# Autodesk Inventor assembly: Assembly7
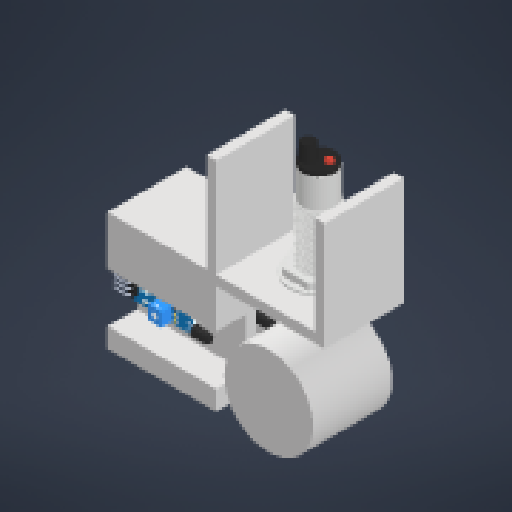
[picture p0: Inventor's stored thumbnail of the model, 512x512]
Saved by Autodesk Inventor 2027.1 (Build 311270010, 270A)
## iProperties
Created: 2026-09-29
Part Number: Assembly7
Document SubType Name: Assembly
Designer: daniel
Author: daniel
## Documents named in this file (5)
- C:\Users\danda\Documents\GitHub\MCT333_Design_of_Mechatronics_Systems_1\CAD\FEED and Sorting\Assembly7.iam
- C:\Users\danda\Documents\GitHub\MCT333_Design_of_Mechatronics_Systems_1\CAD\FEED and Sorting\Part56.ipt
- C:\Users\danda\Documents\GitHub\MCT333_Design_of_Mechatronics_Systems_1\CAD\off_the_shelf_components\18mm-inductive-proximity-sensor-taiss-4\Inductive Proximity Sensor Assembly\Inductive Proximity Sensor Assembly.iam
- C:\Users\danda\Documents\GitHub\MCT333_Design_of_Mechatronics_Systems_1\CAD\off_the_shelf_components\ir-sensor-7.snapshot.2 (1)\IRsensors\IRsensors.iam
- C:\Users\danda\Documents\GitHub\MCT333_Design_of_Mechatronics_Systems_1\CAD\FEED and Sorting\Part23.ipt
## Components (5 placed, 4 different names)
1. Part56:1 — Mate:1, Mate:2, Mate:3, Mate:4, Flush:1
2. Inductive Proximity Sensor Assembly:1 [sub-assembly] — Mate:1, Mate:4, Tangent:1
3. IRsensors:1 [sub-assembly] — Mate:2
4. IRsensors:2 [sub-assembly] — Mate:3
5. Part23:1 — Flush:1, Tangent:1
## Relationships (6: Mate 4, Flush 1, Tangent 1)
- Mate:1: Part56:1 ↔ Inductive Proximity Sensor Assembly:1
- Mate:2: Part56:1 ↔ IRsensors:1
- Mate:3: Part56:1 ↔ IRsensors:2
- Mate:4: Part56:1 ↔ Inductive Proximity Sensor Assembly:1
- Flush:1: Part56:1 ↔ Part23:1
- Tangent:1: Inductive Proximity Sensor Assembly:1 ↔ Part23:1
